# Autodesk Inventor assembly: ASY GBK 2210 short wall shield 4
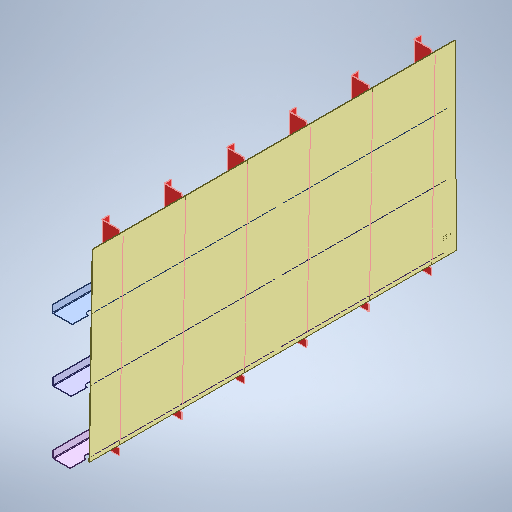
[picture p0: Inventor's stored thumbnail of the model, 512x512]
Saved by Autodesk Inventor 2026 (Build 300175000, 175)
## iProperties
Created: 2026-05-07
Part Number: ASY GBK 2210 short wall shield 4
Document SubType Name: Assembly
Designer: pokla
Stock Number: 1211
Mass: 252568 g
Surface Area: 163192 cm^2
Volume: 32174.3 cm^3
Density: 7.85 g/cm^3
Author: admin
## Documents named in this file (7)
- C:\Users\pokla\Documents\Inventor\GBK-Gubkinskiy\ASY GBK 2210 short wall shield 4.iam
- C:\Users\pokla\Documents\Inventor\GBK-Gubkinskiy\GBK 0101 main rib.ipt
- C:\Users\pokla\Documents\Inventor\GBK-Gubkinskiy\GBK 2211 shield 4.ipt
- C:\Users\pokla\Documents\Inventor\GBK-Gubkinskiy\GBK 0202 stringer 4.ipt
- C:\Users\pokla\Documents\Inventor\GBK-Gubkinskiy\GBK 0203 stringer 5.ipt
- C:\Users\pokla\Documents\Inventor\GBK-Gubkinskiy\GBK 0204 stringer 6.ipt
- C:\Users\pokla\Documents\Inventor\GBK-Gubkinskiy\GBK 0201 second rib.ipt
## Components (13 placed, 5 different names)
1. GBK 0202 stringer 4.ipt:1 — Жесткий:6, Жесткий:1
2. GBK 0202 stringer 4.ipt:2 — Жесткий:1
3. GBK 0203 stringer 5.ipt:1 — Жесткий:5, Жесткий:2
4. GBK 0203 stringer 5.ipt:2 — Жесткий:2
5. GBK 0204 stringer 6.ipt:1 — Жесткий:4, Жесткий:3
6. GBK 0204 stringer 6.ipt:2 — Жесткий:3
7. GBK 2211 shield 4.ipt:1
8. GBK 0201 second rib.ipt:1 — Жесткий:6, Жесткий:5, Жесткий:4
9. GBK 0201 second rib.ipt:2
10. GBK 0201 second rib.ipt:3
11. GBK 0201 second rib.ipt:4
12. GBK 0201 second rib.ipt:5
13. GBK 0201 second rib.ipt:6
## Component patterns: (6 elements, first: GBK 0201 second rib.ipt:1)
## Relationships (6: WeldJoint 6)
- Жесткий:6 [WeldJoint] (4 mm): GBK 0202 stringer 4.ipt:1 ↔ GBK 0201 second rib.ipt:1
- Жесткий:1 [WeldJoint]: GBK 0202 stringer 4.ipt:1 ↔ GBK 0202 stringer 4.ipt:2
- Жесткий:5 [WeldJoint] (4 mm): GBK 0203 stringer 5.ipt:1 ↔ GBK 0201 second rib.ipt:1
- Жесткий:2 [WeldJoint]: GBK 0203 stringer 5.ipt:1 ↔ GBK 0203 stringer 5.ipt:2
- Жесткий:4 [WeldJoint] (4 mm): GBK 0204 stringer 6.ipt:1 ↔ GBK 0201 second rib.ipt:1
- Жесткий:3 [WeldJoint]: GBK 0204 stringer 6.ipt:1 ↔ GBK 0204 stringer 6.ipt:2
## Named parameters: основание_длина_нижнего = 200 mm, основание_длина_верхнего = 100 mm, стрингер_глубина_1 = 190.24693 mm, стрингер_глубина_2 = 178.90614 mm, стрингер_глубина_3 = 167.56536 mm, стрингер_глубина_4 = 156.22457 mm, стрингер_глубина_5 = 144.88379 mm, стрингер_глубина_6 = 133.543 mm, стрингер_глубина_7 = 122.20222 mm, стрингер_глубина_8 = 110.86143 mm, Лист_ширина = 1480 mm, ребро_усилителей = 60 mm, паз_под_стрингер_глубина = 70 mm, паз_под_стрингер_толщина = 5 mm, отступ_от_пола_до_первого_стрингера = 430 mm, шаг_стрингеров = 500 mm, радиус_выреза_под_сварку = 30 mm, нахлест_шпангоутов_1_2 = 150 mm, нахлест_шпангоутов_2_3 = 80 mm, Стрингер_длина = 1490 mm, Лист_длина = 2980 mm, Шаг_шпангоутов = 496.66667 mm
